# Autodesk Inventor assembly: Ensamble bomba
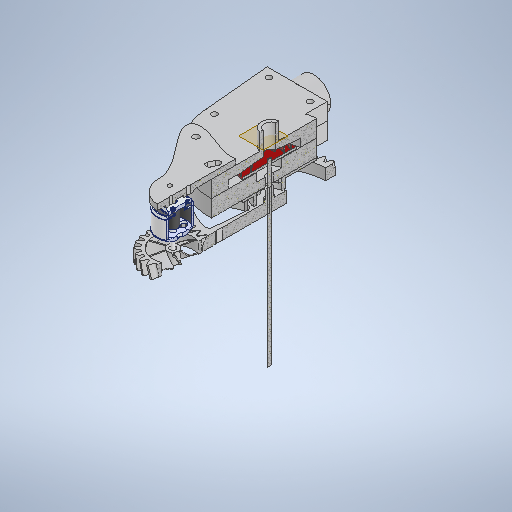
[picture p0: Inventor's stored thumbnail of the model, 512x512]
Saved by Autodesk Inventor 2025.3 (Build 293356000, 356)
## iProperties
Created: 2025-11-12
Part Number: Ensamble bomba
Document SubType Name: Assembly
Designer: juanm
Author: juanm
## Documents named in this file (11)
- C:\Users\juanm\Documents\Inventor\Turbo\Ensamble bomba.iam
- C:\Users\juanm\Documents\Inventor\Turbo\Rodete_4000RPM_2LS.ipt
- C:\Users\juanm\Documents\Inventor\Turbo\Base voluta.ipt
- C:\Users\juanm\Documents\Inventor\Turbo\Tapa voluta.ipt
- C:\Users\juanm\Documents\Inventor\Turbo\Eje 5mm.ipt
- C:\Users\juanm\Documents\Inventor\Turbo\Engrane.ipt
- C:\Users\juanm\Documents\Inventor\Turbo\Motor con soporte\Motor con soporte\Motor con soporte.iam
- C:\Users\juanm\Documents\Inventor\Turbo\Pinon.ipt
- C:\Users\juanm\Documents\Inventor\Turbo\Estructura.ipt
- C:\Users\juanm\Documents\Inventor\Turbo\Soporte motor.ipt
- C:\Users\juanm\Documents\Inventor\Turbo\Anillo rodamiento.ipt
## Components (10 placed, 10 different names)
1. Rodete_4000RPM_2LS:1 — Insert:1, Rotation:1
2. Base voluta:1 — Insert:1, Flush:1, Mate:1, Flush:2, Insert:2, Flush:4, Insert:5
3. Tapa voluta:1 — Flush:1, Mate:1, Flush:2, Flush:5
4. Eje 5mm:1 — Insert:2, Insert:3, Mate:2
5. Engrane:1 — Insert:3, Rotation:1, Rotation:2
6. Pinon:1 — Insert:4, Rotation:2
7. Motor con soporte:1 [sub-assembly] — Mate:2, Insert:4
8. Estructura:1 — Flush:4
9. Soporte motor:1 — Flush:5
10. Anillo rodamiento:1 — Insert:5
## Relationships (13: Insert 5, Flush 4, Mate 2, RelateRotation 2)
- Insert:1 (0.5 mm): Rodete_4000RPM_2LS:1 ↔ Base voluta:1
- Flush:1: Base voluta:1 ↔ Tapa voluta:1
- Mate:1: Base voluta:1 ↔ Tapa voluta:1
- Flush:2: Base voluta:1 ↔ Tapa voluta:1
- Insert:2 (-30 mm): Base voluta:1 ↔ Eje 5mm:1
- Insert:3 (118 mm): Eje 5mm:1 ↔ Engrane:1
- Mate:2 (80 mm): Eje 5mm:1 ↔ Motor con soporte:1
- Insert:4 (9 mm): Pinon:1 ↔ Motor con soporte:1
- Rotation:1 [RelateRotation] (1 ul): Rodete_4000RPM_2LS:1 ↔ Engrane:1
- Rotation:2 [RelateRotation] (2.5 ul): Engrane:1 ↔ Pinon:1
- Flush:4: Base voluta:1 ↔ Estructura:1
- Flush:5: Tapa voluta:1 ↔ Soporte motor:1
- Insert:5: Base voluta:1 ↔ Anillo rodamiento:1
